# Autodesk Inventor assembly: 總組合圖
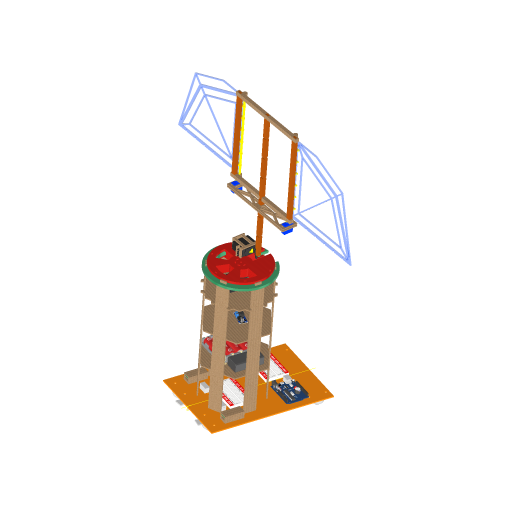
[picture p0: Inventor's stored thumbnail of the model, 512x512]
Saved by Autodesk Inventor 2024 (Build 280153000, 153)
## iProperties
Created: 2024-04-09
Document SubType Name: Assembly
Designer: USER
Mass: 1317.31 g
Surface Area: 9223.84 cm^2
Volume: 1282.93 cm^3
Density: 1.0268 g/cm^3
Author: 第26組
Title: 總組合圖
## Documents named in this file (26)
- C:\Users\op04o\OneDrive\桌面\實務\final\圖檔\DesignVer2_encoder_MG996\DesignVer_final.iam
- C:\Users\op04o\OneDrive\桌面\實務\final\圖檔\DesignVer2_encoder_MG996\cow_wheel.ipt
- C:\Users\op04o\OneDrive\桌面\實務\final\圖檔\DesignVer2_encoder_MG996\back_down_hold.ipt
- C:\Users\op04o\OneDrive\桌面\實務\final\圖檔\DesignVer2_encoder_MG996\middle_space.ipt
- C:\Users\op04o\OneDrive\桌面\實務\final\圖檔\DesignVer2_encoder_MG996\rolling_plate.ipt
- C:\Users\op04o\OneDrive\桌面\實務\final\圖檔\DesignVer2_encoder_MG996\rolling_plate_small.ipt
- C:\Users\op04o\OneDrive\桌面\實務\final\圖檔\DesignVer2_encoder_MG996\sail.iam
- C:\Users\op04o\OneDrive\桌面\實務\final\圖檔\DesignVer2_encoder_MG996\Base_final.ipt
- C:\Users\op04o\OneDrive\桌面\實務\final\圖檔\DesignVer2_encoder_MG996\[3DP]back_cir_hold_final.ipt
- C:\Users\op04o\OneDrive\桌面\實務\final\圖檔\DesignVer2_encoder_MG996\MG996R\MG_996R.iam
- C:\Users\op04o\OneDrive\桌面\實務\final\圖檔\DesignVer2_encoder_MG996\middle_space_3.ipt
- C:\Users\op04o\OneDrive\桌面\實務\final\圖檔\encoder\encoder.iam
- C:\Users\op04o\OneDrive\桌面\實務\final\圖檔\DesignVer2_encoder_MG996\Servo Motor SG90.ipt
- C:\Users\op04o\OneDrive\桌面\實務\final\圖檔\DesignVer2_encoder_MG996\final_circ_plate.ipt
- C:\Users\op04o\OneDrive\桌面\實務\final\圖檔\DesignVer2_encoder_MG996\final_side.ipt
- C:\Users\op04o\OneDrive\桌面\實務\final\圖檔\DesignVer2_encoder_MG996\final_side_hold.ipt
- C:\Users\op04o\OneDrive\桌面\實務\final\圖檔\DesignVer2_encoder_MG996\final_side_hold_2.ipt
- C:\Users\op04o\OneDrive\桌面\實務\final\圖檔\DesignVer2_encoder_MG996\final_side2.ipt
- C:\Users\op04o\OneDrive\桌面\實務\final\圖檔\DesignVer2_encoder_MG996\final_side_hold_3.ipt
- C:\Users\op04o\OneDrive\桌面\實務\final\圖檔\機電設備\18650電池盒\18650電池盒.ipt
- C:\Users\op04o\OneDrive\桌面\實務\final\圖檔\機電設備\Arduino板\Arduino板.iam
- C:\Users\op04o\OneDrive\桌面\實務\final\圖檔\機電設備\麵包板\麵包板.ipt
- C:\Users\op04o\OneDrive\桌面\實務\final\圖檔\機電設備\9V方型電池盒\9V方型電池盒.ipt
- C:\Users\op04o\OneDrive\桌面\實務\final\圖檔\DesignVer2_encoder_MG996\breaker.ipt
- C:\Users\op04o\OneDrive\桌面\實務\final\圖檔\機電設備\lm2596-dc-dc-buck-converter-module-2.snapshot.9\LM2596 DC-DC Buck Converter Module.iam
- LM2596 DC-DC Buck Converter Module.iam
## Components (45 placed, 24 different names)
1. cow_wheel:3 — Mate:80, Mate:81, Mate:85
2. cow_wheel:4 — Mate:75, Mate:76, Mate:77, Mate:78, Mate:79
3. back_down_hold:1 — Mate:99, Mate:100, Mate:101, Mate:102, Mate:107
4. back_down_hold:2 — Flush:14, Flush:28, Mate:92, Mate:93, Mate:94
5. back_down_hold:3 — Flush:5, Mate:47, Flush:13, Mate:90, Mate:91, Mate:108, Mate:138, Mate:139, Mate:140
6. back_down_hold:4 — Mate:87, Mate:97, Mate:98
7. back_down_hold:5 — Flush:6, Mate:46, Flush:12, Mate:48, Mate:88, Mate:89, Mate:105
8. back_down_hold:6 — Flush:5, Flush:6, Mate:95, Mate:96, Mate:109
9. middle_space:1 — Flush:13, Mate:48, Flush:14, Flush:28, Mate:182, Mate:186
10. middle_space:2 — Mate:46, Flush:12, Mate:47, Mate:189
11. rolling_plate:1 — Mate:55, Flush:22, Flush:23, Mate:155
12. rolling_plate:2 — Mate:56, Mate:57, Flush:24, Mate:110
13. rolling_plate_small:1 — Mate:52, Flush:16, Flush:19, Mate:56, Flush:24, Mate:142, Mate:143, Mate:144
14. rolling_plate_small:2 — Mate:52, Mate:53, Flush:16, Flush:17, Flush:19, Flush:20, Mate:57
15. rolling_plate_small:3 — Mate:53, Mate:54, Flush:17, Flush:18, Flush:20, Flush:21, Mate:156, Flush:37
16. rolling_plate_small:4 — Mate:54, Flush:18, Flush:21, Mate:55, Flush:22, Flush:23
17. sail:1 [sub-assembly] — Angle:6, Mate:181, Flush:44
18. Base_final:1 — Mate:75, Mate:76, Mate:77, Mate:78, Mate:79, Mate:80, Mate:81, Mate:85, Mate:87, Mate:88, Mate:89, Mate:90, Mate:91, Mate:92, Mate:93, Mate:94, Mate:95, Mate:96, Mate:97, Mate:98, Mate:99, Mate:100, Mate:101, Mate:102, Mate:105, Mate:115, Mate:116, Mate:117, Mate:118, Mate:131, Mate:134, Angle:2, Angle:4, Flush:29, Mate:145, Mate:146, Mate:147, Mate:148, Mate:149, Mate:151, Mate:152, Mate:153, Angle:5, Flush:33, Flush:34, Flush:35, Flush:36, Mate:154, Mate:183, Mate:184, Mate:185
19. [3DP]back_cir_hold_final:1 — Mate:107, Mate:108, Mate:109, Mate:110, Mate:142
20. cow_wheel:5 — Mate:131, Mate:145, Mate:146, Mate:147
21. cow_wheel:6 — Mate:134, Mate:148, Mate:149
22. MG_996R:1 [sub-assembly] — Angle:2, Mate:141, Mate:143, Mate:144, Angle:6
23. middle_space_3:1 — Mate:138, Mate:139, Mate:140, Mate:141
24. encoder:1 [sub-assembly] — Angle:3, Angle:4, Flush:30, Mate:151, Flush:31, Mate:154
25. encoder:2 [sub-assembly] — Angle:3, Flush:29, Flush:30, Flush:31, Mate:152
26. Servo Motor SG90:1 — Flush:32, Mate:153, Angle:5, Flush:33, Flush:34, Mate:188
27. Servo Motor SG90:2 — Flush:32, Flush:35, Flush:36, Mate:187
28. final_circ_plate:1 — Mate:155, Mate:156, Flush:37, Mate:157, Mate:158, Mate:159, Mate:160, Mate:161, Mate:164, Mate:165, Mate:166, Mate:167, Mate:168, Mate:169, Mate:170, Mate:173, Mate:174, Mate:175
29. MG_996R:2 [sub-assembly] — Mate:157, Mate:171, Mate:172, Mate:181, Flush:44
30. final_side:1 — Mate:164, Mate:165, Mate:169, Mate:176, Flush:39, Mate:177
31. final_side:2 — Mate:166, Mate:167, Mate:168
32. final_side_hold:1 — Mate:176, Flush:39, Mate:177, Mate:178, Flush:41
33. final_side_hold_2:1 — Mate:173, Mate:174, Mate:175, Flush:40, Flush:42, Mate:180
34. final_side2:1 — Mate:158, Mate:159, Mate:170, Flush:38
35. final_side2:2 — Mate:160, Mate:161, Flush:38, Mate:171, Mate:172
36. final_side_hold_3:1 — Flush:40, Flush:43, Mate:180
37. final_side_hold_3:2 — Mate:178, Flush:41, Flush:42, Flush:43
38. 18650電池盒:1 — Mate:182, Flush:45
39. Arduino板:1 [sub-assembly] — Mate:183
40. 麵包板:1 — Mate:184
41. 麵包板:2 — Mate:185
42. 9V方型電池盒:1 — Mate:186, Flush:45
43. breaker:1 — Mate:187
44. breaker:2 — Mate:188
45. LM2596 DC-DC Buck Converter Module:1 [sub-assembly] — Mate:189
## Relationships (131: Mate 94, Flush 32, Angle 5)
- Flush:5: back_down_hold:3 ↔ back_down_hold:6
- Flush:6: back_down_hold:5 ↔ back_down_hold:6
- Mate:46: back_down_hold:5 ↔ middle_space:2
- Flush:12: back_down_hold:5 ↔ middle_space:2
- Mate:47: back_down_hold:3 ↔ middle_space:2
- Flush:13: back_down_hold:3 ↔ middle_space:1
- Mate:48: back_down_hold:5 ↔ middle_space:1
- Flush:14: back_down_hold:2 ↔ middle_space:1
- Mate:52: rolling_plate_small:1 ↔ rolling_plate_small:2
- Mate:53: rolling_plate_small:2 ↔ rolling_plate_small:3
- Mate:54: rolling_plate_small:3 ↔ rolling_plate_small:4
- Flush:16: rolling_plate_small:1 ↔ rolling_plate_small:2
- Flush:17: rolling_plate_small:2 ↔ rolling_plate_small:3
- Flush:18: rolling_plate_small:3 ↔ rolling_plate_small:4
- Flush:19: rolling_plate_small:1 ↔ rolling_plate_small:2
- Flush:20: rolling_plate_small:2 ↔ rolling_plate_small:3
- Flush:21: rolling_plate_small:3 ↔ rolling_plate_small:4
- Mate:55: rolling_plate:1 ↔ rolling_plate_small:4
- Flush:22: rolling_plate:1 ↔ rolling_plate_small:4
- Flush:23: rolling_plate:1 ↔ rolling_plate_small:4
- Mate:56: rolling_plate:2 ↔ rolling_plate_small:1
- Mate:57: rolling_plate:2 ↔ rolling_plate_small:2
- Flush:24: rolling_plate:2 ↔ rolling_plate_small:1
- Flush:28: back_down_hold:2 ↔ middle_space:1
- Mate:75: cow_wheel:4 ↔ Base_final:1
- Mate:76: cow_wheel:4 ↔ Base_final:1
- Mate:77: cow_wheel:4 ↔ Base_final:1
- Mate:78: cow_wheel:4 ↔ Base_final:1
- Mate:79: cow_wheel:4 ↔ Base_final:1
- Mate:80: cow_wheel:3 ↔ Base_final:1
- Mate:81: cow_wheel:3 ↔ Base_final:1
- Mate:85: cow_wheel:3 ↔ Base_final:1
- Mate:87: back_down_hold:4 ↔ Base_final:1
- Mate:88: back_down_hold:5 ↔ Base_final:1
- Mate:89: back_down_hold:5 ↔ Base_final:1
- Mate:90: back_down_hold:3 ↔ Base_final:1
- Mate:91: back_down_hold:3 ↔ Base_final:1
- Mate:92: back_down_hold:2 ↔ Base_final:1
- Mate:93: back_down_hold:2 ↔ Base_final:1
- Mate:94: back_down_hold:2 ↔ Base_final:1
- Mate:95: back_down_hold:6 ↔ Base_final:1
- Mate:96: back_down_hold:6 ↔ Base_final:1
- Mate:97: back_down_hold:4 ↔ Base_final:1
- Mate:98: back_down_hold:4 ↔ Base_final:1
- Mate:99: back_down_hold:1 ↔ Base_final:1
- Mate:100: back_down_hold:1 ↔ Base_final:1
- Mate:101: back_down_hold:1 ↔ Base_final:1
- Mate:102: back_down_hold:1 ↔ Base_final:1
- Mate:105: back_down_hold:5 ↔ Base_final:1
- Mate:107: back_down_hold:1 ↔ [3DP]back_cir_hold_final:1
- Mate:108: back_down_hold:3 ↔ [3DP]back_cir_hold_final:1
- Mate:109: back_down_hold:6 ↔ [3DP]back_cir_hold_final:1
- Mate:110 (0.5 mm): rolling_plate:2 ↔ [3DP]back_cir_hold_final:1
- Mate:115: Base_final:1
- Mate:116: Base_final:1
- Mate:117: Base_final:1
- Mate:118: Base_final:1
- Mate:119
- Mate:120
- Mate:131: Base_final:1 ↔ cow_wheel:5
- Mate:134: Base_final:1 ↔ cow_wheel:6
- Angle:2 (0 deg): Base_final:1 ↔ MG_996R:1
- Mate:138: back_down_hold:3 ↔ middle_space_3:1
- Mate:139: back_down_hold:3 ↔ middle_space_3:1
- Mate:140: back_down_hold:3 ↔ middle_space_3:1
- Mate:141: MG_996R:1 ↔ middle_space_3:1
- Mate:142: rolling_plate_small:1 ↔ [3DP]back_cir_hold_final:1
- Mate:143: rolling_plate_small:1 ↔ MG_996R:1
- Mate:144: rolling_plate_small:1 ↔ MG_996R:1
- Angle:3 (0 deg): encoder:1 ↔ encoder:2
- Angle:4 (0 deg): Base_final:1 ↔ encoder:1
- Flush:29 (-12 mm): Base_final:1 ↔ encoder:2
- Flush:30: encoder:1 ↔ encoder:2
- Mate:145: Base_final:1 ↔ cow_wheel:5
- Mate:146: Base_final:1 ↔ cow_wheel:5
- Mate:147: Base_final:1 ↔ cow_wheel:5
- Mate:148: Base_final:1 ↔ cow_wheel:6
- Mate:149: Base_final:1 ↔ cow_wheel:6
- Mate:151 (0.1 mm): Base_final:1 ↔ encoder:1
- Flush:31: encoder:1 ↔ encoder:2
- Mate:152 (0.1 mm): Base_final:1 ↔ encoder:2
- Flush:32: Servo Motor SG90:1 ↔ Servo Motor SG90:2
- Mate:153: Base_final:1 ↔ Servo Motor SG90:1
- Angle:5 (0 deg): Base_final:1 ↔ Servo Motor SG90:1
- Flush:33 (55 mm): Base_final:1 ↔ Servo Motor SG90:1
- Flush:34 (55 mm): Base_final:1 ↔ Servo Motor SG90:1
- Flush:35 (55 mm): Base_final:1 ↔ Servo Motor SG90:2
- Flush:36 (55 mm): Base_final:1 ↔ Servo Motor SG90:2
- Mate:154 (0.1 mm): Base_final:1 ↔ encoder:1
- Mate:155: rolling_plate:1 ↔ final_circ_plate:1
- Mate:156: rolling_plate_small:3 ↔ final_circ_plate:1
- Flush:37: rolling_plate_small:3 ↔ final_circ_plate:1
- Mate:157: final_circ_plate:1 ↔ MG_996R:2
- Mate:158: final_circ_plate:1 ↔ final_side2:1
- Mate:159: final_circ_plate:1 ↔ final_side2:1
- Mate:160: final_circ_plate:1 ↔ final_side2:2
- Mate:161: final_circ_plate:1 ↔ final_side2:2
- Mate:164: final_circ_plate:1 ↔ final_side:1
- Mate:165: final_circ_plate:1 ↔ final_side:1
- Mate:166: final_circ_plate:1 ↔ final_side:2
- Mate:167: final_circ_plate:1 ↔ final_side:2
- Mate:168: final_circ_plate:1 ↔ final_side:2
- Mate:169: final_circ_plate:1 ↔ final_side:1
- Mate:170: final_circ_plate:1 ↔ final_side2:1
- Flush:38: final_side2:1 ↔ final_side2:2
- Mate:171: MG_996R:2 ↔ final_side2:2
- Mate:172: MG_996R:2 ↔ final_side2:2
- Mate:173: final_circ_plate:1 ↔ final_side_hold_2:1
- Mate:174: final_circ_plate:1 ↔ final_side_hold_2:1
- Mate:175: final_circ_plate:1 ↔ final_side_hold_2:1
- Mate:176: final_side:1 ↔ final_side_hold:1
- Flush:39: final_side:1 ↔ final_side_hold:1
- Mate:177: final_side:1 ↔ final_side_hold:1
- Flush:40: final_side_hold_2:1 ↔ final_side_hold_3:1
- Mate:178: final_side_hold:1 ↔ final_side_hold_3:2
- Flush:41: final_side_hold:1 ↔ final_side_hold_3:2
- Flush:42: final_side_hold_2:1 ↔ final_side_hold_3:2
- Flush:43: final_side_hold_3:1 ↔ final_side_hold_3:2
- Mate:180: final_side_hold_2:1 ↔ final_side_hold_3:1
- Angle:6 (-90 deg): sail:1 ↔ MG_996R:1
- Mate:181: sail:1 ↔ MG_996R:2
- Flush:44: sail:1 ↔ MG_996R:2
- Mate:182: middle_space:1 ↔ 18650電池盒:1
- Mate:183: Base_final:1 ↔ Arduino板:1
- Mate:184: Base_final:1 ↔ 麵包板:1
- Mate:185: Base_final:1 ↔ 麵包板:2
- Mate:186: middle_space:1 ↔ 9V方型電池盒:1
- Flush:45: 18650電池盒:1 ↔ 9V方型電池盒:1
- Mate:187: Servo Motor SG90:2 ↔ breaker:1
- Mate:188: Servo Motor SG90:1 ↔ breaker:2
- Mate:189: middle_space:2 ↔ LM2596 DC-DC Buck Converter Module:1
